# Autodesk Inventor assembly: climber-assy
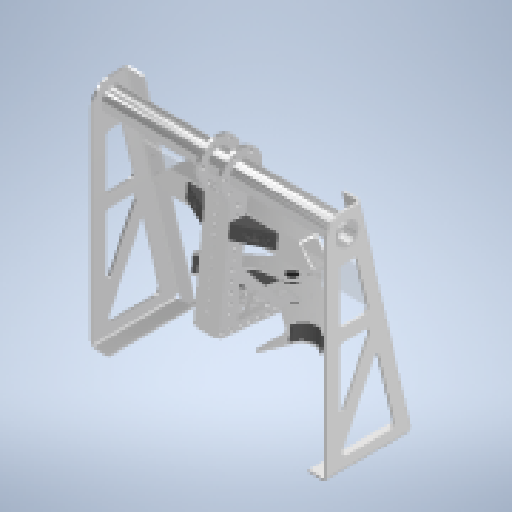
[picture p0: Inventor's stored thumbnail of the model, 512x512]
Saved by Autodesk Inventor 2025.2 (Build 292293000, 293)
## iProperties
Category: _
Manager: _
ILogicPurgeVersion: 0.0.0.0
OnSaveVersion: 3.2.6.0
OnSaveAssembly: COREAutomationManager
Created: 2025-03-18
Part Number: climber-assy
Checked By: 00
Engr Approved By: _
User Status: Work In Process
Description: ASSY,STANDARD (mm)
Document SubType Name: Assembly
Mfg Approved By: Paul.Struhar
Designer: mathe
Mass: 1430.47 g
Surface Area: 3969 cm^2
Volume: 594.124 cm^3
CN_MASS: 0
CN_SERVICEABLE: _
FIRST_DESCRIPTION: _
SECOND_DESCRIPTION: _
THIRD_DESCRIPTION: _
CL_runCount: 0
ModelCat: Uncategorized
Subject: _
Author: mathe
Keywords: -
Revision Number: A
## Documents named in this file (6)
- C:\Users\Baz Robotics\Downloads\2025-Poseidon-Mechanical\climber-assy.iam
- C:\Users\Baz Robotics\Downloads\2025-Poseidon-Mechanical\Climber support.ipt
- C:\Users\Baz Robotics\Downloads\2025-Poseidon-Mechanical\Climber support_MIR.ipt
- C:\Users\Baz Robotics\Downloads\2025-Poseidon-Mechanical\climber-axle.ipt
- C:\Users\Baz Robotics\Downloads\2025-Poseidon-Mechanical\grapplinghook.iam
- C:\Users\Baz Robotics\Documents\Climber lexan back piece.ipt
## Components (5 placed, 5 different names)
1. Climber support:1 — Mate:1, Flush:1, Mate:2, Flush:2, Flush:3, Mate:3, Insert:1, Insert:2, Mate:5
2. Climber support_MIR:1 — Flush:2, Flush:3, Mate:3, Mate:6, Mate:7
3. climber-axle:1 — Insert:1
4. grapplinghook:1 [sub-assembly] — Insert:2
5. Climber lexan back piece:1 — Mate:5, Mate:6, Mate:7
## Relationships (11: Mate 6, Flush 3, Insert 2)
- Mate:1: Climber support:1
- Flush:1: Climber support:1
- Mate:2: Climber support:1
- Flush:2: Climber support:1 ↔ Climber support_MIR:1
- Flush:3: Climber support:1 ↔ Climber support_MIR:1
- Mate:3 (325.12 mm): Climber support:1 ↔ Climber support_MIR:1
- Insert:1 (-40.64 mm): Climber support:1 ↔ climber-axle:1
- Insert:2 (145.0975 mm): Climber support:1 ↔ grapplinghook:1
- Mate:5: Climber support:1 ↔ Climber lexan back piece:1
- Mate:6 (100 mm): Climber support_MIR:1 ↔ Climber lexan back piece:1
- Mate:7 (3.81 mm): Climber support_MIR:1 ↔ Climber lexan back piece:1
